# Autodesk Inventor assembly: StressTest
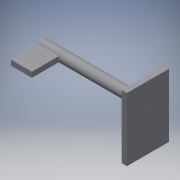
[picture p0: Inventor's stored thumbnail of the model, 180x180]
Saved by Autodesk Inventor 2017 (Build 210142000, 142)
## iProperties
Created: 2018-03-21
Part Number: StressTest
Document SubType Name: Assembly
Designer: User
Mass: 45.0296 g
Surface Area: 167.412 cm^2
Volume: 45.0296 cm^3
Density: 1 g/cm^3
Author: User
## Documents named in this file (11)
- C:\Robotics\CAD\2018-19_CAD\StressTest.iam
- C:\Robotics\CAD\2018-19_CAD\Offseason\StressTestPart.ipt
- C:\Robotics\CAD\2018-19_CAD\Offseason\StressTestPlate.ipt
- C:\Robotics\CAD\2018-19_CAD\StressTest\AIP\FEA\cghwi1e0w.fins
- C:\Robotics\CAD\2018-19_CAD\StressTest\AIP\FEA\cghwi1e0w.fsat
- C:\Robotics\CAD\2018-19_CAD\StressTest\AIP\FEA\cghwi1e0w.ftes
- C:\Robotics\CAD\2018-19_CAD\StressTest\AIP\FEA\cghwi1e0w.fwiz
- C:\Robotics\CAD\2018-19_CAD\StressTest\AIP\FEA\cghwi1e2o.fmsh
- C:\Robotics\CAD\2018-19_CAD\StressTest\AIP\FEA\cghwi1e2p.fres
- C:\Robotics\CAD\2018-19_CAD\StressTest\AIP\FEA\cgkfbvra8.fmsh
- C:\Robotics\CAD\2018-19_CAD\StressTest\AIP\FEA\cgkfbvra9.fres
## Components (2 placed, 2 different names)
1. StressTestPart:1 — Mate:1, Insert:1
2. StressTestPlate:1 — Mate:1, Insert:1
## Relationships (2: Mate 1, Insert 1)
- Mate:1: StressTestPart:1 ↔ StressTestPlate:1
- Insert:1: StressTestPart:1 ↔ StressTestPlate:1
## Named parameters: sa_0 = 4519.39
note: some values were not read from the file. Shown as the stored number, unit unknown: "sa_0".
